# Autodesk Inventor assembly: Stop System Assembly
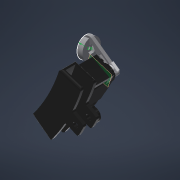
[picture p0: Inventor's stored thumbnail of the model, 180x180]
Saved by Autodesk Inventor 2021 (Build 250183000, 183)
## iProperties
RuleStatus: InUse
Created: 2020-12-21
Vendor: HHMI: JRC - ID&F
Document SubType Name: Assembly
Designer: winnubstj
AfterDocSave0: file://Part Number Cleaner
DESIGN DEPARTMENT: HHMI: JRC - ID&F
ALTERED ITEM PART NUMBER: N/A
ALTERED ITEM VENDOR: N/A
ALTERED ITEM DESCRIPTION: N/A
Author: winnubstj
Revision Number: 0
## Documents named in this file (7)
- Y:\repos\vr-ball-lock\Inventor Models\Stop System Assembly.iam
- Y:\repos\vr-ball-lock\Inventor Models\Parts\16 inch ball treadmill frame v2.ipt
- Y:\repos\vr-ball-lock\Inventor Models\Parts\Frame Holder.ipt
- Y:\repos\vr-ball-lock\Inventor Models\Parts\hs-422_sws.ipt
- Y:\repos\vr-ball-lock\Inventor Models\Parts\servo connector.ipt
- Y:\repos\vr-ball-lock\Inventor Models\Parts\base de riel.ipt
- Y:\repos\vr-ball-lock\Inventor Models\Parts\arm.ipt
## Components (6 placed, 6 different names)
1. 16 inch ball treadmill frame v2:1 — Mate:1, Mate:2
2. Frame Holder:1 — Mate:1, Mate:2, Rigid:1
3. hs-422_sws:1 — Rigid:1, Rotational:1
4. servo connector:1
5. base de riel:1 — Rotational:1, Slider:3
6. arm:1 — Slider:3
## Relationships (5: Mate 2, WeldJoint 1, RevoluteJoint 1, TranslationJoint 1)
- Mate:1: 16 inch ball treadmill frame v2:1 ↔ Frame Holder:1
- Mate:2: 16 inch ball treadmill frame v2:1 ↔ Frame Holder:1
- Rigid:1 [WeldJoint] (4 mm): Frame Holder:1 ↔ hs-422_sws:1
- Rotational:1 [RevoluteJoint]: hs-422_sws:1 ↔ base de riel:1
- Slider:3 [TranslationJoint]: base de riel:1 ↔ arm:1
